# Autodesk Inventor assembly: sub_leg_1_lit
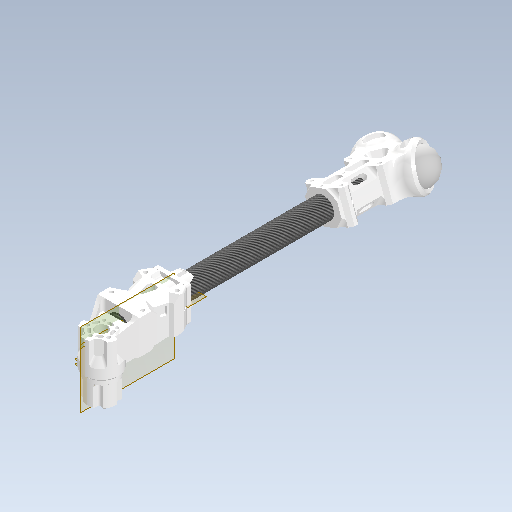
[picture p0: Inventor's stored thumbnail of the model, 512x512]
Saved by Autodesk Inventor 2020 (Build 240168000, 168)
## iProperties
Created: 2020-09-02
Part Number: sub_leg_1_lit
Document SubType Name: Assembly
Designer: psrobotics
Author: psrobotics
## Documents named in this file (6)
- D:\projects-3\biped_gen1\hardware\sub_leg_1_lit.iam
- D:\projects-3\biped_gen1\hardware\joint_connector_5_lit.ipt
- D:\projects-3\biped_gen1\hardware\carbon_fiber_25_21_300.ipt
- D:\projects-3\biped_gen1\hardware\joint_connector_6.ipt
- D:\projects-3\biped_gen1\hardware\foot_ass.iam
- D:\projects-3\biped_gen1\hardware\joint_connector_4_str.ipt
## Components (5 placed, 5 different names)
1. joint_connector_5_lit:1 — Insert:7, Insert:8, Insert:10, Insert:11
2. carbon_fiber_25_21_300:1 — Insert:6, Insert:9
3. joint_connector_6:1 — Insert:10, Insert:11
4. foot_ass:1 [sub-assembly] — Insert:6, Angle:1
5. joint_connector_4_str:1 — Insert:7, Insert:8, Insert:9, Angle:1
## Relationships (7: Insert 6, Angle 1)
- Insert:6: carbon_fiber_25_21_300:1 ↔ foot_ass:1
- Insert:7: joint_connector_5_lit:1 ↔ joint_connector_4_str:1
- Insert:8: joint_connector_5_lit:1 ↔ joint_connector_4_str:1
- Insert:9: carbon_fiber_25_21_300:1 ↔ joint_connector_4_str:1
- Insert:10: joint_connector_5_lit:1 ↔ joint_connector_6:1
- Insert:11: joint_connector_5_lit:1 ↔ joint_connector_6:1
- Angle:1 (-20 deg): foot_ass:1 ↔ joint_connector_4_str:1
